# Autodesk Inventor assembly: Assembly_3_master
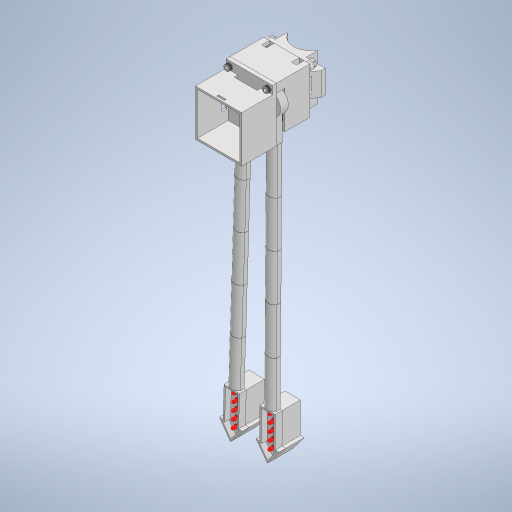
[picture p0: Inventor's stored thumbnail of the model, 512x512]
Saved by Autodesk Inventor 2023 (Build 270158000, 158)
## iProperties
Created: 2023-09-30
Part Number: Assembly_3_master
Document SubType Name: Assembly
Designer: zskus
Author: zskus
## Documents named in this file (6)
- C:\Users\zskus\Desktop\Folders\Personal Projects\Inventor\Project_1_Scooter\Assembly\Assembly_3_master.iam
- C:\Users\zskus\Desktop\Folders\Personal Projects\Inventor\Project_1_Scooter\Parts\Part_4_scooter_attachment.ipt
- C:\Users\zskus\Desktop\Folders\Personal Projects\Inventor\Project_1_Scooter\Assembly\Assembly_2_servobox.iam
- C:\Users\zskus\Desktop\Folders\Personal Projects\Inventor\Project_1_Scooter\Parts\Part_1_box.ipt
- C:\Users\zskus\Desktop\Folders\Personal Projects\Inventor\Project_1_Scooter\Parts\90044A425_Black-Oxide Alloy Steel Socket Head Screw.ipt
- C:\Users\zskus\Desktop\Folders\Personal Projects\Inventor\Project_1_Scooter\Parts\95462A029_Medium-Strength Steel Hex Nut.ipt
## Components (7 placed, 5 different names)
1. Part_4_scooter_attachment:1 — Mate:1, Mate:6, Mate:7, Mate:9, Mate:15, Mate:16
2. Assembly_2_servobox:1 [sub-assembly] — Mate:1, Mate:2, Mate:7, Mate:8, Mate:10
3. Part_1_box:1 — Mate:2, Mate:8, Mate:9, Mate:10, Mate:11, Mate:12, Mate:13, Mate:14
4. 90044A425_Black-Oxide Alloy Steel Socket Head Screw:1 — Mate:5, Mate:11, Mate:12
5. 95462A029_Medium-Strength Steel Hex Nut:1 — Mate:5, Mate:6
6. 90044A425_Black-Oxide Alloy Steel Socket Head Screw:2 — Mate:13, Mate:14
7. 95462A029_Medium-Strength Steel Hex Nut:2 — Mate:15, Mate:16
## Relationships (14: Mate 14)
- Mate:1: Part_4_scooter_attachment:1 ↔ Assembly_2_servobox:1
- Mate:2: Assembly_2_servobox:1 ↔ Part_1_box:1
- Mate:5: 90044A425_Black-Oxide Alloy Steel Socket Head Screw:1 ↔ 95462A029_Medium-Strength Steel Hex Nut:1
- Mate:6: Part_4_scooter_attachment:1 ↔ 95462A029_Medium-Strength Steel Hex Nut:1
- Mate:7: Part_4_scooter_attachment:1 ↔ Assembly_2_servobox:1
- Mate:8: Assembly_2_servobox:1 ↔ Part_1_box:1
- Mate:9: Part_4_scooter_attachment:1 ↔ Part_1_box:1
- Mate:10: Assembly_2_servobox:1 ↔ Part_1_box:1
- Mate:11: Part_1_box:1 ↔ 90044A425_Black-Oxide Alloy Steel Socket Head Screw:1
- Mate:12: Part_1_box:1 ↔ 90044A425_Black-Oxide Alloy Steel Socket Head Screw:1
- Mate:13: Part_1_box:1 ↔ 90044A425_Black-Oxide Alloy Steel Socket Head Screw:2
- Mate:14: Part_1_box:1 ↔ 90044A425_Black-Oxide Alloy Steel Socket Head Screw:2
- Mate:15: Part_4_scooter_attachment:1 ↔ 95462A029_Medium-Strength Steel Hex Nut:2
- Mate:16: Part_4_scooter_attachment:1 ↔ 95462A029_Medium-Strength Steel Hex Nut:2
